# Autodesk Inventor assembly: Assembly2タミヤダンパー　下
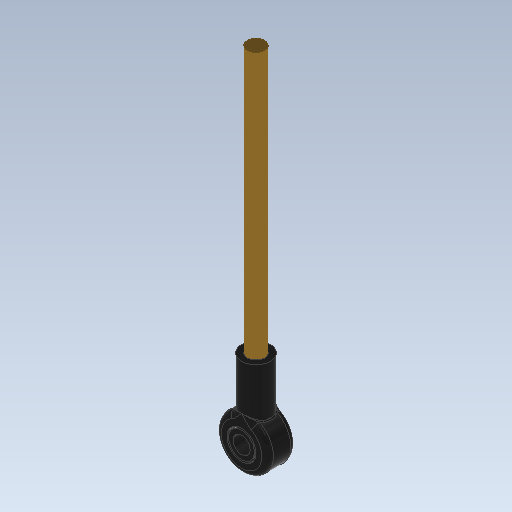
[picture p0: Inventor's stored thumbnail of the model, 512x512]
Saved by Autodesk Inventor 2020.2 (Build 242310000, 310)
## iProperties
Created: 2018-09-18
Part Number: Assembly2タミヤダンパー　下
Material: 一般
Document SubType Name: Assembly
Designer: 杉本　賢二郎
Author: 杉本　賢二郎
## Documents named in this file (4)
- C:\Users\aoyam\Desktop\SRDC_local\Inventor\二年機\Geminiβ\汎用部品\ダンパー\Assembly2タミヤダンパー　下.iam
- C:\Users\aoyam\Desktop\SRDC_local\Inventor\二年機\Geminiβ\汎用部品\ダンパー\タミヤダンパー部品5.ipt
- C:\Users\aoyam\Desktop\SRDC_local\Inventor\二年機\Geminiβ\汎用部品\ダンパー\タミヤダンパー部品7.ipt
- C:\Users\aoyam\Desktop\SRDC_local\Inventor\二年機\Geminiβ\汎用部品\ダンパー\タミヤダンパー部品8.ipt
## Components (3 placed, 3 different names)
1. タミヤダンパー部品5:1 — 挿入:2
2. タミヤダンパー部品7:1 — 挿入:1, 挿入:2
3. タミヤダンパー部品8:1 — 挿入:1
## Relationships (2: Insert 2)
- 挿入:1 [Insert]: タミヤダンパー部品7:1 ↔ タミヤダンパー部品8:1
- 挿入:2 [Insert] (-3 mm): タミヤダンパー部品5:1 ↔ タミヤダンパー部品7:1
